# Autodesk Inventor assembly: Guida con supporto
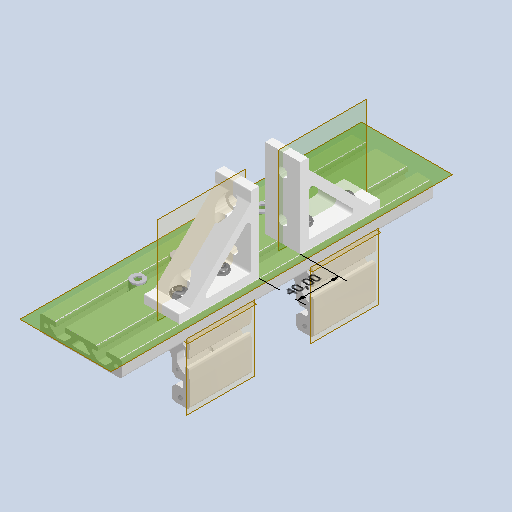
[picture p0: Inventor's stored thumbnail of the model, 512x512]
Saved by Autodesk Inventor 2022 (Build 260153000, 153)
## iProperties
RuleStatus: InUse
Created: 2021-12-29
Part Number: Guida con supporto
Document SubType Name: Assembly
Designer: matte
Author: matte
## Documents named in this file (7)
- C:\Users\matte\Documents\GitHub\MDM-CyberOrto-CAD\Pezzi singoli\Supporto lineare\Guida con supporto.iam
- C:\Users\matte\Documents\GitHub\MDM-CyberOrto-CAD\Pezzi singoli\Supporto lineare\Piastra-supporto.ipt
- C:\Users\matte\Documents\GitHub\MDM-CyberOrto-CAD\Parker components\08-Linear Application\06-Linear Roller System\01-Roller System 6\30-401.ipt
- C:\Users\matte\Documents\GitHub\MDM-CyberOrto-CAD\Parker components\03-Brackets_Gussets_Plates\09-Machined Gussets\20-102.ipt
- C:\Users\matte\Documents\GitHub\MDM-CyberOrto-CAD\Parker components\02-Fasteners\16-Screws\01-Metric Screws\01-Button Head\24-145-8.ipt
- C:\Users\matte\Documents\GitHub\MDM-CyberOrto-CAD\Parker components\02-Fasteners\10-Standard T-Nuts\20-050.ipt
- C:\Users\matte\Documents\GitHub\MDM-CyberOrto-CAD\Pezzi singoli\Supporto lineare\Doppia Giuntura.iam
## Components (15 placed, 6 different names)
1. Piastra-supporto:1 — Coincidente:1, Coincidente:2, Coincidente:3, Coincidente:4, Allineato:1, Allineato:2, Coincidente:5, Coincidente:6, Allineato:3, Coincidente:7, Allineato:4, Coincidente:19, Allineato:5, Coincidente:20, Coincidente:21, Allineato:6, Coincidente:25, Allineato:7, Coincidente:26, Allineato:9, Coincidente:27, Coincidente:28, Coincidente:30, Coincidente:31
2. Doppia Giuntura:2 [sub-assembly] — Coincidente:30, Coincidente:31, Coincidente:32
3. 30-401:1 — Coincidente:4, Allineato:1, Coincidente:13, Coincidente:24, Allineato:8
4. 20-102:1 — Coincidente:5, Coincidente:6, Allineato:3, Coincidente:8, Coincidente:9, Coincidente:10
5. 24-145-8:1 — Coincidente:7, Coincidente:8, Coincidente:11
6. 24-145-8:2 — Coincidente:9, Coincidente:10, Coincidente:12
7. 20-050:1 — Coincidente:11, Coincidente:12, Coincidente:13
8. 30-401:2 — Allineato:4, Coincidente:19, Coincidente:23, Coincidente:24, Allineato:10
9. 20-102:2 — Coincidente:22, Allineato:6
10. 24-145-8:3 — Coincidente:21, Coincidente:22
11. 24-145-8:4 — Coincidente:20
12. 20-050:2 — Coincidente:23
13. Doppia Giuntura:1 [sub-assembly] — Coincidente:27, Coincidente:28, Coincidente:29
14. 30-401:3 — Coincidente:25, Allineato:7, Allineato:8, Coincidente:32
15. 30-401:4 — Coincidente:26, Allineato:9, Allineato:10, Coincidente:29
## Relationships (42: Mate 32, Flush 10)
- Coincidente:1 [Mate]: Piastra-supporto:1
- Coincidente:2 [Mate]: Piastra-supporto:1
- Coincidente:3 [Mate]: Piastra-supporto:1
- Coincidente:4 [Mate]: Piastra-supporto:1 ↔ 30-401:1
- Allineato:1 [Flush]: Piastra-supporto:1 ↔ 30-401:1
- Allineato:2 [Flush]: Piastra-supporto:1
- Coincidente:5 [Mate]: Piastra-supporto:1 ↔ 20-102:1
- Coincidente:6 [Mate]: Piastra-supporto:1 ↔ 20-102:1
- Allineato:3 [Flush]: Piastra-supporto:1 ↔ 20-102:1
- Coincidente:7 [Mate]: Piastra-supporto:1 ↔ 24-145-8:1
- Coincidente:8 [Mate]: 20-102:1 ↔ 24-145-8:1
- Coincidente:9 [Mate]: 20-102:1 ↔ 24-145-8:2
- Coincidente:10 [Mate]: 20-102:1 ↔ 24-145-8:2
- Coincidente:11 [Mate]: 24-145-8:1 ↔ 20-050:1
- Coincidente:12 [Mate]: 24-145-8:2 ↔ 20-050:1
- Coincidente:13 [Mate]: 30-401:1 ↔ 20-050:1
- [Mate]: 20-102:2 ↔ 24-145-8:3
- [Mate]: 20-102:2 ↔ 24-145-8:4
- [Mate]: 20-102:2 ↔ 24-145-8:4
- [Mate]: 24-145-8:3 ↔ 20-050:2
- [Mate]: 24-145-8:4 ↔ 20-050:2
- Allineato:4 [Flush]: Piastra-supporto:1 ↔ 30-401:2
- Coincidente:19 [Mate]: Piastra-supporto:1 ↔ 30-401:2
- Allineato:5 [Flush]: Piastra-supporto:1
- Coincidente:20 [Mate]: Piastra-supporto:1 ↔ 24-145-8:4
- Coincidente:21 [Mate]: Piastra-supporto:1 ↔ 24-145-8:3
- Coincidente:22 [Mate]: 20-102:2 ↔ 24-145-8:3
- Allineato:6 [Flush]: Piastra-supporto:1 ↔ 20-102:2
- Coincidente:23 [Mate]: 30-401:2 ↔ 20-050:2
- Coincidente:24 [Mate] (60 mm): 30-401:1 ↔ 30-401:2
- Coincidente:25 [Mate]: Piastra-supporto:1 ↔ 30-401:3
- Allineato:7 [Flush]: Piastra-supporto:1 ↔ 30-401:3
- Allineato:8 [Flush]: 30-401:1 ↔ 30-401:3
- Coincidente:26 [Mate]: Piastra-supporto:1 ↔ 30-401:4
- Allineato:9 [Flush]: Piastra-supporto:1 ↔ 30-401:4
- Allineato:10 [Flush]: 30-401:2 ↔ 30-401:4
- Coincidente:27 [Mate]: Piastra-supporto:1 ↔ Doppia Giuntura:1
- Coincidente:28 [Mate]: Piastra-supporto:1 ↔ Doppia Giuntura:1
- Coincidente:29 [Mate]: Doppia Giuntura:1 ↔ 30-401:4
- Coincidente:30 [Mate]: Piastra-supporto:1 ↔ Doppia Giuntura:2
- Coincidente:31 [Mate]: Piastra-supporto:1 ↔ Doppia Giuntura:2
- Coincidente:32 [Mate]: Doppia Giuntura:2 ↔ 30-401:3
## Named parameters: L_piastra = 300 mm, d54_d52 = 0 mm, d55_d48 = 0 mm, d56_d49 = 0 mm, d57_d50 = 0 mm, d58_d51 = 0 mm
